# Autodesk Inventor assembly: Shifter v1
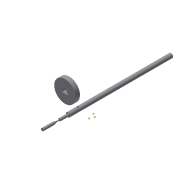
[picture p0: Inventor's stored thumbnail of the model, 180x180]
Saved by Autodesk Inventor 2014 (Build 180170000, 170)
## iProperties
Created: 2014-02-23
Part Number: Shifter v1
Document SubType Name: Assembly
Designer: Owner
Author: Owner
## Documents named in this file (5)
- C:\Users\Owner\Documents\Inventor\FRC 2014\Frc Chassis 2014\Shifter v1.iam
- C:\Users\Owner\Documents\Inventor\FRC 2014\Frc Chassis 2014\transmission plunger.ipt
- C:\Users\Owner\Documents\Inventor\FRC 2014\Frc Chassis 2014\augmented gear v3.ipt
- C:\Users\Owner\Documents\Inventor\FRC 2014\Frc Chassis 2014\Ball bearing - .1875.ipt
- C:\Users\Owner\Documents\Inventor\FRC 2014\Frc Chassis 2014\transmission tube v1.ipt
## Components (6 placed, 4 different names)
1. transmission plunger:1 — Insert:1
2. augmented gear v3:1
3. Ball bearing - .1875:1
4. Ball bearing - .1875:2
5. Ball bearing - .1875:3
6. transmission tube v1:1 — Insert:1
## Relationships (1: Insert 1)
- Insert:1: transmission plunger:1 ↔ transmission tube v1:1
